# Autodesk Inventor assembly: SideSensor
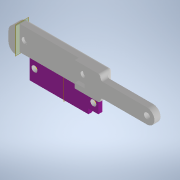
[picture p0: Inventor's stored thumbnail of the model, 180x180]
Saved by Autodesk Inventor 2022 (Build 260153000, 153)
## iProperties
Created: 2022-09-16
Part Number: SideSensor
Document SubType Name: Assembly
Designer: Yazawa
Author: Yazawa
## Documents named in this file (3)
- C:\Users\Yazawa\Documents\GitHub\murakumo\inventor\SideSensor.iam
- C:\Users\Yazawa\Documents\GitHub\murakumo\inventor\SideSensorCircuit_MIR1.ipt
- C:\Users\Yazawa\Documents\GitHub\murakumo\inventor\SideSensor_Mount.ipt
## Components (2 placed, 2 different names)
1. SideSensor_Mount:1 — フラッシュ:1, フラッシュ:2, フラッシュ:3
2. SideSensorCircuit_MIR1:1 — フラッシュ:1, フラッシュ:2, フラッシュ:3
## Relationships (3: Flush 3)
- フラッシュ:1 [Flush]: SideSensor_Mount:1 ↔ SideSensorCircuit_MIR1:1
- フラッシュ:2 [Flush]: SideSensor_Mount:1 ↔ SideSensorCircuit_MIR1:1
- フラッシュ:3 [Flush]: SideSensor_Mount:1 ↔ SideSensorCircuit_MIR1:1
